# Autodesk Inventor assembly: ASSY_CLAMPING_RING
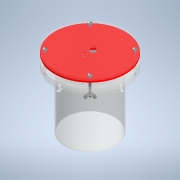
[picture p0: Inventor's stored thumbnail of the model, 180x180]
Saved by Autodesk Inventor 2021 (Build 250183000, 183)
## iProperties
Company: CHAROSA
Created: 2020-09-01
Part Number: ASSY_CLAMPING_RING
Document SubType Name: Assembly
Designer: C. SULLIVAN
Project: BIOLUMEN REACTOR
Checked By: C. SULLIVAN
Engr Approved By: C. SULLIVAN
Description: ACRYLIC CLAMPING RING W/ GASKET
Mfg Approved By: C. SULLIVAN
Engineer: C. SULLIVAN
Author: C. SULLIVAN
Title: SUB-ASSY, CLAMPING RING W_BEAKER
Revision Number: A
## Documents named in this file (10)
- C:\Users\Public\Documents\BioLumen Reactor\V2\Inventor_Versions\ASSY_CLAMPING_RING.iam
- C:\Users\Public\Documents\BioLumen Reactor\V2\Inventor_Versions\UPPERRING.ipt
- C:\Users\Public\Documents\BioLumen Reactor\V2\Inventor_Versions\GASKET.ipt
- C:\Users\Public\Documents\BioLumen Reactor\V2\Inventor_Versions\LOWERRING1.ipt
- C:\Users\Public\Documents\BioLumen Reactor\V2\Inventor_Versions\LOWERRING2.ipt
- C:\Users\Public\Documents\BioLumen Reactor\V2\Inventor_Versions\LOWERRING3.ipt
- C:\Users\Public\Documents\BioLumen Reactor\V2\Inventor_Versions\PLASTIC_LATCH.ipt
- C:\Users\Public\Documents\BioLumen Reactor\V2\Inventor_Versions\SIMPLE_BEAKER.ipt
- C:\Users\Conor\Documents\Inventor\Content Center Files\R2021\en-US\SS-EN-ISO 7045  H\EN ISO 7045 - M4 x 40H.ipt
- C:\Users\Conor\Documents\Inventor\Content Center Files\R2021\en-US\KS B 1014\KS B 1014 - M 4.ipt
## Components (18 placed, 9 different names)
1. UPPERRING — Insert:1, Insert:2, Insert:3, Insert:4
2. GASKET
3. LOWERRING1 — Mate:1
4. LOWERRING2 — Mate:1, Mate:2
5. LOWERRING3 — Mate:2, Mate:10
6. PLASTIC_LATCH
7. PLASTIC_LATCH:1
8. PLASTIC_LATCH:2
9. PLASTIC_LATCH:3
10. SIMPLE_BEAKER
11. SS EN ISO 7045 H M4 x 40:1 — Insert:1
12. SS EN ISO 7045 H M4 x 40:2 — Insert:2
13. SS EN ISO 7045 H M4 x 40:3 — Insert:3, Mate:9
14. SS EN ISO 7045 H M4 x 40:4 — Insert:4
15. KS B 1014 - Metric M 4:1 — Mate:9, Mate:10
16. KS B 1014 - Metric M 4:2
17. KS B 1014 - Metric M 4:3
18. KS B 1014 - Metric M 4:4
## Relationships (14: Mate 10, Insert 4)
- Mate:1: LOWERRING1 ↔ LOWERRING2
- Mate:2: LOWERRING2 ↔ LOWERRING3
- Insert:1: UPPERRING ↔ SS EN ISO 7045 H M4 x 40:1
- Insert:2: UPPERRING ↔ SS EN ISO 7045 H M4 x 40:2
- Insert:3: UPPERRING ↔ SS EN ISO 7045 H M4 x 40:3
- Insert:4: UPPERRING ↔ SS EN ISO 7045 H M4 x 40:4
- [Mate]: SS EN ISO 7045 H M4 x 40:2 ↔ KS B 1014 - Metric M 4:4
- [Mate]: LOWERRING3 ↔ KS B 1014 - Metric M 4:4
- [Mate]: SS EN ISO 7045 H M4 x 40:4 ↔ KS B 1014 - Metric M 4:3
- [Mate]: LOWERRING3 ↔ KS B 1014 - Metric M 4:3
- Mate:9: SS EN ISO 7045 H M4 x 40:3 ↔ KS B 1014 - Metric M 4:1
- Mate:10: LOWERRING3 ↔ KS B 1014 - Metric M 4:1
- [Mate]: SS EN ISO 7045 H M4 x 40:1 ↔ KS B 1014 - Metric M 4:2
- [Mate]: LOWERRING3 ↔ KS B 1014 - Metric M 4:2
